# Autodesk Inventor assembly: Electrical Board - back top
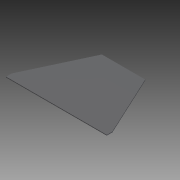
[picture p0: Inventor's stored thumbnail of the model, 180x180]
Saved by Autodesk Inventor 2012 (Build 160160000, 160)
## iProperties
Created: 2012-01-15
Part Number: Electrical Board - back top
Document SubType Name: Assembly
Designer: Antonella Wilby
Author: Antonella Wilby
## Documents named in this file (3)
- C:\Users\Antonella\Documents\GCC Robotics 2012 - Mechanical\Robot 2.0\Electrical\Back Electrical Board\Top\Electrical Board - back top.iam
- C:\Users\Antonella\Documents\GCC Robotics 2012 - Mechanical\Robot 2.0\Electrical\Back Electrical Board\Top\Electrical Board - back top.ipt
- C:\Users\Antonella\Documents\GCC Robotics 2012 - Mechanical\Robot 2.0\Electrical\Back Electrical Board\top board mount bracket.ipt
## Components (3 placed, 2 different names)
1. Electrical Board - back top:1 — Mate:1, Mate:2, Flush:1, Mate:5
2. top board mount bracket:1 — Mate:2, Mate:3, Mate:4, Flush:1, Mate:5
3. top board mount bracket:2 — Mate:1, Mate:3, Mate:4
## Relationships (6: Mate 5, Flush 1)
- Mate:1: Electrical Board - back top:1 ↔ top board mount bracket:2
- Mate:2: Electrical Board - back top:1 ↔ top board mount bracket:1
- Mate:3: top board mount bracket:1 ↔ top board mount bracket:2
- Mate:4 (254 mm): top board mount bracket:1 ↔ top board mount bracket:2
- Flush:1 (-76.2 mm): Electrical Board - back top:1 ↔ top board mount bracket:1
- Mate:5 (127 mm): Electrical Board - back top:1 ↔ top board mount bracket:1
